# Autodesk Inventor assembly: BaseBoxAssembly
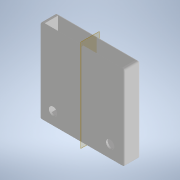
[picture p0: Inventor's stored thumbnail of the model, 180x180]
Saved by Autodesk Inventor 2022 (Build 260153000, 153)
## iProperties
Created: 2022-08-24
Part Number: BaseBoxAssembly
Document SubType Name: Assembly
Designer: sgioj
Author: sgioj
## Documents named in this file (3)
- C:\Autodesk\wirelessLights\BaseBoxAssembly.iam
- C:\Autodesk\wirelessLights\BaseBox.ipt
- C:\Autodesk\wirelessLights\baseHook.ipt
## Components (3 placed, 2 different names)
1. BaseBox:1 — Mate:1, Mate:2, Flush:1, Mate:3, Angle:1, Mate:4, Mate:5, Flush:2
2. baseHook:1 — Mate:1, Mate:2, Flush:1
3. baseHook:2 — Mate:4, Mate:5, Flush:2
## Relationships (8: Mate 5, Flush 2, Angle 1)
- Mate:1 (-2.4 mm): BaseBox:1 ↔ baseHook:1
- Mate:2 (0.2 mm): BaseBox:1 ↔ baseHook:1
- Flush:1 (17.393 mm): BaseBox:1 ↔ baseHook:1
- Mate:3: BaseBox:1
- Angle:1 (0 deg): BaseBox:1
- Mate:4 (0.2 mm): BaseBox:1 ↔ baseHook:2
- Mate:5 (-2.4 mm): BaseBox:1 ↔ baseHook:2
- Flush:2 (17.393 mm): BaseBox:1 ↔ baseHook:2
